# Autodesk Inventor assembly: HeadUnit
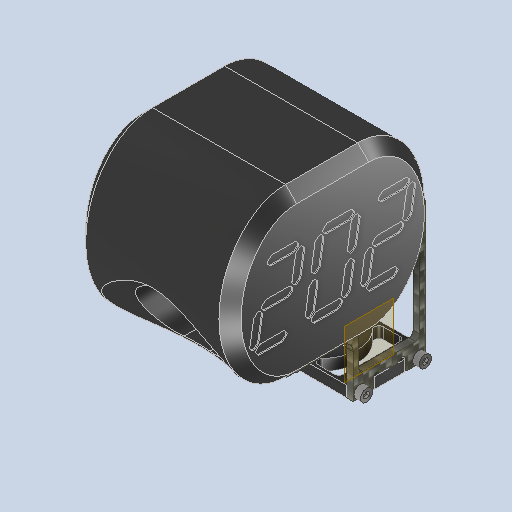
[picture p0: Inventor's stored thumbnail of the model, 512x512]
Saved by Autodesk Inventor 2024.2 (Build 282272000, 272)
## iProperties
Created: 2024-01-19
Part Number: HeadUnit
Document SubType Name: Assembly
Designer: Masato Kubotera
Mass: 275.737 g
Surface Area: 1059.57 cm^2
Volume: 211.056 cm^3
Density: 1.30646 g/cm^3
Author: Masato Kubotera
## Documents named in this file (19)
- C:\Users\masato\OneDrive - Chiba Institute of Technology\CIT Brains\RoboCup2024\Mechanic\SUSTAINA-OP2\NativeFiles\Boby\Head\HeadUnit.iam
- C:\Users\masato\OneDrive - Chiba Institute of Technology\CIT Brains\RoboCup2024\Mechanic\SUSTAINA-OP2\NativeFiles\Boby\COTS\Screws\CapScrew\UC-0308.ipt
- C:\Users\masato\OneDrive - Chiba Institute of Technology\CIT Brains\RoboCup2024\Mechanic\SUSTAINA-OP2\NativeFiles\Boby\Head\HeadCameraMountFrame.ipt
- C:\Users\masato\OneDrive - Chiba Institute of Technology\CIT Brains\RoboCup2024\Mechanic\SUSTAINA-OP2\NativeFiles\Boby\Head\HeadHornFrame.ipt
- C:\Users\masato\OneDrive - Chiba Institute of Technology\CIT Brains\RoboCup2024\Mechanic\SUSTAINA-OP2\NativeFiles\Boby\Head\HeadSideFrame.ipt
- C:\Users\masato\OneDrive - Chiba Institute of Technology\CIT Brains\RoboCup2024\Mechanic\SUSTAINA-OP2\NativeFiles\Boby\COTS\Spacers\C-2006-4.ipt
- C:\Users\masato\OneDrive - Chiba Institute of Technology\CIT Brains\RoboCup2024\Mechanic\SUSTAINA-OP2\NativeFiles\Boby\Head\HeadSpeakerMountFrame.ipt
- C:\Users\masato\OneDrive - Chiba Institute of Technology\CIT Brains\RoboCup2024\Mechanic\SUSTAINA-OP2\NativeFiles\Boby\COTS\ElectronicComponents\CMS-402811-28SP.ipt
- C:\Users\masato\OneDrive - Chiba Institute of Technology\CIT Brains\RoboCup2024\Mechanic\SUSTAINA-OP2\NativeFiles\Boby\Head\HeadCircuitMountFrame.ipt
- C:\Users\masato\OneDrive - Chiba Institute of Technology\CIT Brains\RoboCup2024\Mechanic\SUSTAINA-OP2\NativeFiles\Boby\COTS\Screws\CapScrew\UC-0206.ipt
- C:\Users\masato\OneDrive - Chiba Institute of Technology\CIT Brains\RoboCup2024\Mechanic\SUSTAINA-OP2\NativeFiles\Boby\Head\HeadCover.ipt
- C:\Users\masato\OneDrive - Chiba Institute of Technology\CIT Brains\RoboCup2024\Mechanic\SUSTAINA-OP2\NativeFiles\Boby\COTS\ElectronicComponents\Cameras\e-CAM50_CUONX.ipt
- C:\Users\masato\OneDrive - Chiba Institute of Technology\CIT Brains\RoboCup2024\Mechanic\SUSTAINA-OP2\NativeFiles\Boby\COTS\Spacers\C-2002.5-4.ipt
- C:\Users\masato\OneDrive - Chiba Institute of Technology\CIT Brains\RoboCup2024\Mechanic\SUSTAINA-OP2\NativeFiles\Boby\COTS\Screws\CapScrew\FC-0215EB.ipt
- C:\Users\masato\OneDrive - Chiba Institute of Technology\CIT Brains\RoboCup2024\Mechanic\SUSTAINA-OP2\NativeFiles\Boby\CustomElectronicComponents\SUSTAINA-USB-AUDIO-BOARD.ipt
- C:\Users\masato\OneDrive - Chiba Institute of Technology\CIT Brains\RoboCup2024\Mechanic\SUSTAINA-OP2\NativeFiles\Boby\CustomElectronicComponents\SUSTAINA-SCI-TO-HDMI-BOARD.ipt
- C:\Users\masato\OneDrive - Chiba Institute of Technology\CIT Brains\RoboCup2024\Mechanic\SUSTAINA-OP2\NativeFiles\Boby\COTS\Spacers\BRU-2006S.ipt
- C:\Users\masato\OneDrive - Chiba Institute of Technology\CIT Brains\RoboCup2024\Mechanic\SUSTAINA-OP2\NativeFiles\Boby\COTS\Screws\CapScrew\UC-0204.ipt
- C:\Users\masato\OneDrive - Chiba Institute of Technology\CIT Brains\RoboCup2024\Mechanic\SUSTAINA-OP2\NativeFiles\Boby\COTS\CIL926-F2.4-M12A650.ipt
## Components (57 placed, 18 different names)
1. C-2002.5-4:1 — Insert:93, Insert:116
2. C-2002.5-4:2 — Insert:92, Insert:117
3. C-2002.5-4:3
4. C-2002.5-4:4
5. SUSTAINA-USB-AUDIO-BOARD:1 — Insert:102, Insert:103, Insert:104, Insert:105, Insert:106, Insert:107
6. SUSTAINA-SCI-TO-HDMI-BOARD:1 — Insert:94, Insert:95, Insert:96, Insert:97
7. UC-0206:15 — Insert:96
8. UC-0206:16 — Insert:97
9. BRU-2006S:1 — Insert:98, Insert:102
10. BRU-2006S:2 — Insert:99, Insert:103
11. BRU-2006S:3 — Insert:100
12. BRU-2006S:4 — Insert:101
13. UC-0204:1 — Insert:104
14. UC-0204:2 — Insert:105
15. UC-0204:3 — Insert:106
16. UC-0204:4 — Insert:107
17. CIL926-F2.4-M12A650:1 — Insert:118
18. e-CAM50_CUONX:1 — Insert:108, Insert:109, Insert:110, Insert:111, Insert:112, Insert:113, Insert:114, Insert:115, Insert:116, Insert:117, Insert:118
19. HeadSpeakerMountFrame:1 — Insert:58, Insert:59, Insert:66, Insert:67, Insert:68, Insert:69
20. HeadCircuitMountFrame:1 — Insert:74, Insert:75, Insert:94, Insert:95, Insert:98, Insert:99, Insert:100, Insert:101
21. HeadCameraMountFrame:1 — Insert:37, Insert:38, Insert:92, Insert:93
22. HeadSideFrame:1 — Insert:29, Insert:30, Insert:31, Insert:32, Insert:37, Insert:38, Insert:42, Insert:43, Insert:58, Insert:59, Insert:62, Insert:63, Insert:74, Insert:75, Insert:82, Insert:83
23. HeadSideFrame:2 — Insert:33, Insert:34, Insert:35, Insert:36
24. HeadHornFrame:1 — Mate:1, Angle:1, Mate:2, Insert:24, Insert:25, Insert:26, Insert:29, Insert:30, Insert:33, Insert:34
25. HeadCover:1
26. CMS-402811-28SP:1 — Insert:66, Insert:67, Insert:68, Insert:69, Insert:70, Insert:71, Insert:72, Insert:73
27. FC-0215EB:1 — Insert:108
28. FC-0215EB:2 — Insert:110
29. FC-0215EB:3 — Insert:112
30. FC-0215EB:4 — Insert:114
31. UC-0308:1 — Insert:31
32. UC-0308:2 — Insert:32
33. UC-0308:3 — Insert:36
34. UC-0308:4 — Insert:35
35. UC-0308:6 — Insert:24
36. UC-0308:7 — Insert:25
37. UC-0308:8 — Insert:26
38. UC-0308:9 — Insert:70
39. UC-0308:10 — Insert:71
40. UC-0308:11 — Insert:72
41. UC-0308:12 — Insert:73
42. UC-0206:3 — Insert:42
43. UC-0206:4 — Insert:43
44. UC-0206:5 — Insert:62
45. UC-0206:6 — Insert:63
46. UC-0206:7
47. UC-0206:8
48. UC-0206:9
49. UC-0206:10
50. UC-0206:11 — Insert:82
51. UC-0206:12 — Insert:83
52. UC-0206:13
53. UC-0206:14
54. C-2006-4:1 — Insert:109
55. C-2006-4:2 — Insert:113
56. C-2006-4:3 — Insert:111
57. C-2006-4:4 — Insert:115
## Relationships (76: Insert 70, Flush 3, Mate 2, Angle 1)
- Mate:1: HeadHornFrame:1
- Angle:1 (0 deg): HeadHornFrame:1
- Mate:2: HeadHornFrame:1
- Insert:24: HeadHornFrame:1 ↔ UC-0308:6
- Insert:25: HeadHornFrame:1 ↔ UC-0308:7
- Insert:26: HeadHornFrame:1 ↔ UC-0308:8
- Insert:29: HeadSideFrame:1 ↔ HeadHornFrame:1
- Insert:30: HeadSideFrame:1 ↔ HeadHornFrame:1
- Insert:31: HeadSideFrame:1 ↔ UC-0308:1
- Insert:32: HeadSideFrame:1 ↔ UC-0308:2
- Insert:33: HeadSideFrame:2 ↔ HeadHornFrame:1
- Insert:34: HeadSideFrame:2 ↔ HeadHornFrame:1
- Insert:35: HeadSideFrame:2 ↔ UC-0308:4
- Insert:36: HeadSideFrame:2 ↔ UC-0308:3
- Insert:37: HeadCameraMountFrame:1 ↔ HeadSideFrame:1
- Insert:38: HeadCameraMountFrame:1 ↔ HeadSideFrame:1
- [Insert]: HeadCameraMountFrame:1 ↔ HeadSideFrame:2
- [Insert]: HeadCameraMountFrame:1 ↔ HeadSideFrame:2
- Insert:42: HeadSideFrame:1 ↔ UC-0206:3
- Insert:43: HeadSideFrame:1 ↔ UC-0206:4
- [Insert]: HeadSideFrame:2 ↔ UC-0206:7
- [Insert]: HeadSideFrame:2 ↔ UC-0206:8
- [Flush]: HeadCover:1
- [Flush]: HeadCover:1
- [Flush]: HeadCover:1
- Insert:58: HeadSpeakerMountFrame:1 ↔ HeadSideFrame:1
- Insert:59: HeadSpeakerMountFrame:1 ↔ HeadSideFrame:1
- [Insert]: HeadSpeakerMountFrame:1 ↔ HeadSideFrame:2
- [Insert]: HeadSpeakerMountFrame:1 ↔ HeadSideFrame:2
- Insert:62: HeadSideFrame:1 ↔ UC-0206:5
- Insert:63: HeadSideFrame:1 ↔ UC-0206:6
- [Insert]: HeadSideFrame:2 ↔ UC-0206:9
- [Insert]: HeadSideFrame:2 ↔ UC-0206:10
- Insert:66: HeadSpeakerMountFrame:1 ↔ CMS-402811-28SP:1
- Insert:67: HeadSpeakerMountFrame:1 ↔ CMS-402811-28SP:1
- Insert:68: HeadSpeakerMountFrame:1 ↔ CMS-402811-28SP:1
- Insert:69: HeadSpeakerMountFrame:1 ↔ CMS-402811-28SP:1
- Insert:70: CMS-402811-28SP:1 ↔ UC-0308:9
- Insert:71: CMS-402811-28SP:1 ↔ UC-0308:10
- Insert:72: CMS-402811-28SP:1 ↔ UC-0308:11
- Insert:73: CMS-402811-28SP:1 ↔ UC-0308:12
- Insert:74: HeadCircuitMountFrame:1 ↔ HeadSideFrame:1
- Insert:75: HeadCircuitMountFrame:1 ↔ HeadSideFrame:1
- [Insert]: HeadCircuitMountFrame:1 ↔ HeadSideFrame:2
- [Insert]: HeadCircuitMountFrame:1 ↔ HeadSideFrame:2
- Insert:82: HeadSideFrame:1 ↔ UC-0206:11
- Insert:83: HeadSideFrame:1 ↔ UC-0206:12
- [Insert]: HeadSideFrame:2 ↔ UC-0206:13
- [Insert]: HeadSideFrame:2 ↔ UC-0206:14
- Insert:92: C-2002.5-4:2 ↔ HeadCameraMountFrame:1
- Insert:93: C-2002.5-4:1 ↔ HeadCameraMountFrame:1
- Insert:94: SUSTAINA-SCI-TO-HDMI-BOARD:1 ↔ HeadCircuitMountFrame:1
- Insert:95: SUSTAINA-SCI-TO-HDMI-BOARD:1 ↔ HeadCircuitMountFrame:1
- Insert:96: SUSTAINA-SCI-TO-HDMI-BOARD:1 ↔ UC-0206:15
- Insert:97: SUSTAINA-SCI-TO-HDMI-BOARD:1 ↔ UC-0206:16
- Insert:98: BRU-2006S:1 ↔ HeadCircuitMountFrame:1
- Insert:99: BRU-2006S:2 ↔ HeadCircuitMountFrame:1
- Insert:100: BRU-2006S:3 ↔ HeadCircuitMountFrame:1
- Insert:101: BRU-2006S:4 ↔ HeadCircuitMountFrame:1
- Insert:102: SUSTAINA-USB-AUDIO-BOARD:1 ↔ BRU-2006S:1
- Insert:103: SUSTAINA-USB-AUDIO-BOARD:1 ↔ BRU-2006S:2
- Insert:104: SUSTAINA-USB-AUDIO-BOARD:1 ↔ UC-0204:1
- Insert:105: SUSTAINA-USB-AUDIO-BOARD:1 ↔ UC-0204:2
- Insert:106: SUSTAINA-USB-AUDIO-BOARD:1 ↔ UC-0204:3
- Insert:107: SUSTAINA-USB-AUDIO-BOARD:1 ↔ UC-0204:4
- Insert:108: e-CAM50_CUONX:1 ↔ FC-0215EB:1
- Insert:109: e-CAM50_CUONX:1 ↔ C-2006-4:1
- Insert:110: e-CAM50_CUONX:1 ↔ FC-0215EB:2
- Insert:111: e-CAM50_CUONX:1 ↔ C-2006-4:3
- Insert:112: e-CAM50_CUONX:1 ↔ FC-0215EB:3
- Insert:113: e-CAM50_CUONX:1 ↔ C-2006-4:2
- Insert:114: e-CAM50_CUONX:1 ↔ FC-0215EB:4
- Insert:115: e-CAM50_CUONX:1 ↔ C-2006-4:4
- Insert:116: C-2002.5-4:1 ↔ e-CAM50_CUONX:1
- Insert:117: C-2002.5-4:2 ↔ e-CAM50_CUONX:1
- Insert:118 (-8 mm): CIL926-F2.4-M12A650:1 ↔ e-CAM50_CUONX:1
